# Autodesk Inventor assembly: ToolAssambly2
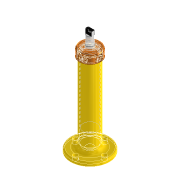
[picture p0: Inventor's stored thumbnail of the model, 180x180]
Saved by Autodesk Inventor 2021 (Build 250183000, 183)
## iProperties
Created: 2022-09-01
Part Number: ToolAssambly2
Document SubType Name: Assembly
Designer: brian
Author: brian
## Documents named in this file (4)
- G:\Mi unidad\Universidad\Control\Robotica\Laboratorio\ToolAssambly2.iam
- G:\Mi unidad\Universidad\Control\Robotica\Laboratorio\Marker.ipt
- G:\Mi unidad\Universidad\Control\Robotica\Laboratorio\Tool.ipt
- G:\Mi unidad\Universidad\Control\Robotica\Laboratorio\ToolCap.ipt
## Components (3 placed, 3 different names)
1. Marker:1 — Cylindrical:1
2. Tool:1 — Mate:1, Mate:2, Flush:1, Rotational:1, Cylindrical:1
3. ToolCap:1 — Rotational:1
## Relationships (5: Mate 2, Flush 1, RevoluteJoint 1, CylindricalJoint 1)
- Mate:1: Tool:1
- Mate:2: Tool:1
- Flush:1: Tool:1
- Rotational:1 [RevoluteJoint]: Tool:1 ↔ ToolCap:1
- Cylindrical:1: Marker:1 ↔ Tool:1
